# Autodesk Inventor assembly: Framing_For_Roof
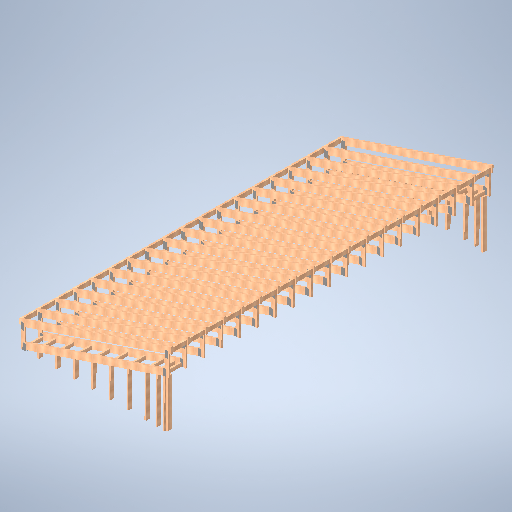
[picture p0: Inventor's stored thumbnail of the model, 512x512]
Saved by Autodesk Inventor 2025.1 (Build 291241020, 241B)
## iProperties
Created: 2024-10-03
Part Number: Framing_For_Roof
Document SubType Name: Assembly
Designer: Tom
Author: Tom
## Documents named in this file (17)
- C:\Users\Tom\Documents\Inventor\Mobility\Additional_Building\Framing_For_Roof.iam
- C:\Users\Tom\Documents\Inventor\Mobility\Additional_Building\Truss.iam
- C:\Users\Tom\Documents\Inventor\Mobility\Additional_Building\Stud_With_Height_5.047_Inches.ipt
- C:\Users\Tom\Documents\Inventor\Mobility\Additional_Building\Stud_With_Height_10.386_Inches.ipt
- C:\Users\Tom\Documents\Inventor\Mobility\Additional_Building\Stud_With_Height_15.724_Inches.ipt
- C:\Users\Tom\Documents\Inventor\Mobility\Additional_Building\Stud_With_Height_21.063_Inches.ipt
- C:\Users\Tom\Documents\Inventor\Mobility\Additional_Building\Stud_With_Height_26.401_Inches.ipt
- C:\Users\Tom\Documents\Inventor\Mobility\Additional_Building\Stud_With_Height_31.740_Inches.ipt
- C:\Users\Tom\Documents\Inventor\Mobility\Additional_Building\Stud_With_Height_37.078_Inches.ipt
- C:\Users\Tom\Documents\Inventor\Mobility\Additional_Building\Stud_With_Height_40.373_Inches.ipt
- C:\Users\Tom\Documents\Inventor\Mobility\Additional_Building\Stud_With_Height_42.5_Inches.ipt
- C:\Users\Tom\Documents\Inventor\Mobility\Additional_Building\Stud_With_Height_42.5_Inches_And_Cut.ipt
- C:\Users\Tom\Documents\Inventor\Mobility\Additional_Building\Subfascia_With_Dimensions_4.023_x_13.75_Inches.ipt
- C:\Users\Tom\Documents\Inventor\Mobility\Additional_Building\Subfascia_With_Dimensions_4.023_x_14.5_Inches.ipt
- C:\Users\Tom\Documents\Inventor\Mobility\Additional_Building\Subfascia_With_Dimensions_3.725_x_13.75_Inches.ipt
- C:\Users\Tom\Documents\Inventor\Mobility\Additional_Building\Subfascia_With_Dimensions_3.725_x_14.5_Inches.ipt
- C:\Users\Tom\Documents\Inventor\Mobility\Additional_Building\Support_For_Ceiling.ipt
## Components (95 placed, 16 different names)
1. Subfascia_With_Dimensions_4.023_x_13.75_Inches:1 — Mate:5, Flush:30, Flush:31
2. Subfascia_With_Dimensions_4.023_x_13.75_Inches:2 — Mate:7, Flush:35, Flush:36
3. Subfascia_With_Dimensions_3.725_x_13.75_Inches:1 — Mate:8, Flush:37, Flush:38
4. Subfascia_With_Dimensions_3.725_x_13.75_Inches:2 — Mate:10, Flush:41, Flush:42
5. Truss:1 [sub-assembly] — Mate:10, Flush:41, Flush:42
6. Truss:2 [sub-assembly] — Flush:1, Flush:2, Flush:3, Flush:4, Flush:5, Flush:6, Flush:8, Flush:9, Flush:11, Flush:12, Flush:14, Flush:15, Flush:17, Flush:18, Flush:20, Flush:21, Flush:23, Flush:24, Flush:26, Mate:2, Flush:28, Mate:3, Mate:5, Flush:30, Flush:31, Flush:32, Mate:11, Flush:44, Mate:12, Mate:13, Flush:46, Mate:14, Flush:48, Mate:15, Flush:50, Mate:16, Flush:52, Mate:17, Flush:54, Mate:18, Flush:56, Mate:19, Flush:58, Mate:20, Flush:60, Mate:21, Flush:62, Flush:65
7. Truss:3 [sub-assembly] — Flush:1, Flush:2, Flush:32, Mate:6, Flush:33, Flush:34, Mate:8, Flush:37, Flush:38
8. Truss:4 [sub-assembly] — Mate:9, Flush:39, Flush:40
9. Truss:5 [sub-assembly]
10. Truss:6 [sub-assembly]
11. Truss:7 [sub-assembly]
12. Truss:8 [sub-assembly]
13. Truss:9 [sub-assembly]
14. Truss:10 [sub-assembly]
15. Truss:11 [sub-assembly]
16. Truss:12 [sub-assembly]
17. Truss:13 [sub-assembly]
18. Truss:14 [sub-assembly]
19. Truss:15 [sub-assembly]
20. Truss:16 [sub-assembly]
21. Truss:17 [sub-assembly]
22. Truss:18 [sub-assembly]
23. Truss:19 [sub-assembly] — Mate:7, Flush:35, Flush:36
24. Subfascia_With_Dimensions_4.023_x_14.5_Inches:1 — Mate:6, Flush:33, Flush:34
25. Subfascia_With_Dimensions_4.023_x_14.5_Inches:2
26. Subfascia_With_Dimensions_4.023_x_14.5_Inches:3
27. Subfascia_With_Dimensions_4.023_x_14.5_Inches:4
28. Subfascia_With_Dimensions_4.023_x_14.5_Inches:5
29. Subfascia_With_Dimensions_4.023_x_14.5_Inches:6
30. Subfascia_With_Dimensions_4.023_x_14.5_Inches:7
31. Subfascia_With_Dimensions_4.023_x_14.5_Inches:8
32. Subfascia_With_Dimensions_4.023_x_14.5_Inches:9
33. Subfascia_With_Dimensions_4.023_x_14.5_Inches:10
34. Subfascia_With_Dimensions_4.023_x_14.5_Inches:11
35. Subfascia_With_Dimensions_4.023_x_14.5_Inches:12
36. Subfascia_With_Dimensions_4.023_x_14.5_Inches:13
37. Subfascia_With_Dimensions_4.023_x_14.5_Inches:14
38. Subfascia_With_Dimensions_4.023_x_14.5_Inches:15
39. Subfascia_With_Dimensions_4.023_x_14.5_Inches:16
40. Subfascia_With_Dimensions_3.725_x_14.5_Inches:1 — Mate:9, Flush:39, Flush:40
41. Subfascia_With_Dimensions_3.725_x_14.5_Inches:2
42. Subfascia_With_Dimensions_3.725_x_14.5_Inches:3
43. Subfascia_With_Dimensions_3.725_x_14.5_Inches:4
44. Subfascia_With_Dimensions_3.725_x_14.5_Inches:5
45. Subfascia_With_Dimensions_3.725_x_14.5_Inches:6
46. Subfascia_With_Dimensions_3.725_x_14.5_Inches:7
47. Subfascia_With_Dimensions_3.725_x_14.5_Inches:8
48. Subfascia_With_Dimensions_3.725_x_14.5_Inches:9
49. Subfascia_With_Dimensions_3.725_x_14.5_Inches:10
50. Subfascia_With_Dimensions_3.725_x_14.5_Inches:11
51. Subfascia_With_Dimensions_3.725_x_14.5_Inches:12
52. Subfascia_With_Dimensions_3.725_x_14.5_Inches:13
53. Subfascia_With_Dimensions_3.725_x_14.5_Inches:14
54. Subfascia_With_Dimensions_3.725_x_14.5_Inches:15
55. Subfascia_With_Dimensions_3.725_x_14.5_Inches:16
56. Support_For_Ceiling:1 — Mate:11, Flush:44, Mate:12
57. Support_For_Ceiling:2 — Mate:13, Flush:45, Flush:46
58. Support_For_Ceiling:3 — Mate:14, Flush:47, Flush:48
59. Support_For_Ceiling:4 — Mate:15, Flush:49, Flush:50
60. Support_For_Ceiling:5 — Mate:16, Flush:51, Flush:52
61. Support_For_Ceiling:6 — Mate:17, Flush:53, Flush:54
62. Support_For_Ceiling:7 — Mate:18, Flush:55, Flush:56
63. Support_For_Ceiling:8 — Mate:19, Flush:57, Flush:58
64. Support_For_Ceiling:9 — Mate:20, Flush:59, Flush:60
65. Support_For_Ceiling:10 — Mate:21, Flush:61, Flush:62
66. Support_For_Ceiling:11
67. Support_For_Ceiling:12
68. Support_For_Ceiling:13
69. Support_For_Ceiling:14
70. Support_For_Ceiling:15
71. Support_For_Ceiling:16
72. Support_For_Ceiling:17
73. Support_For_Ceiling:18
74. Support_For_Ceiling:19
75. Support_For_Ceiling:20
76. Stud_With_Height_5.047_Inches:1 — Flush:3, Flush:4, Flush:5, Flush:7, Flush:45
77. Stud_With_Height_10.386_Inches:1 — Flush:6, Flush:7, Flush:8, Flush:10, Flush:47
78. Stud_With_Height_15.724_Inches:1 — Flush:9, Flush:10, Flush:11, Flush:13, Flush:49
79. Stud_With_Height_21.063_Inches:1 — Flush:12, Flush:13, Flush:14, Flush:16, Flush:51
80. Stud_With_Height_26.401_Inches:1 — Flush:15, Flush:16, Flush:17, Flush:19, Flush:53
81. Stud_With_Height_31.740_Inches:1 — Flush:18, Flush:19, Flush:20, Flush:22, Flush:55
82. Stud_With_Height_37.078_Inches:1 — Flush:21, Flush:22, Flush:23, Flush:25, Flush:57
83. Stud_With_Height_40.373_Inches:1 — Flush:24, Flush:25, Flush:26, Flush:59, Flush:63
84. Stud_With_Height_42.5_Inches_And_Cut:1 — Mate:2, Flush:28, Mate:4, Flush:61, Flush:64, Flush:65
85. Stud_With_Height_5.047_Inches:2
86. Stud_With_Height_10.386_Inches:2
87. Stud_With_Height_15.724_Inches:2
88. Stud_With_Height_21.063_Inches:2
89. Stud_With_Height_26.401_Inches:2
90. Stud_With_Height_31.740_Inches:2
91. Stud_With_Height_37.078_Inches:2
92. Stud_With_Height_40.373_Inches:2
93. Stud_With_Height_42.5_Inches_And_Cut:2
94. Stud_With_Height_42.5_Inches:1 — Mate:3, Mate:4, Flush:63, Flush:64
95. Stud_With_Height_42.5_Inches:2
## Component patterns: (2 elements, first: Truss:1), (17 elements, first: Truss:3), (16 elements, first: Subfascia_With_Dimensions_4.023_x_14.5_Inches:1), (16 elements, first: Subfascia_With_Dimensions_3.725_x_14.5_Inches:1), (2 elements, first: Support_For_Ceiling:1 + Support_For_Ceiling:2 + Support_For_Ceiling:3 + Support_For_Ceiling:4 + Support_For_Ceiling:5 + Support_For_Ceiling:6 + Support_For_Ceiling:7 + Support_For_Ceiling:8 + Support_For_Ceiling:9 + Support_For_Ceiling:10), (2 elements, first: Stud_With_Height_5.047_Inches:1 + Stud_With_Height_10.386_Inches:1 + Stud_With_Height_15.724_Inches:1 + Stud_With_Height_21.063_Inches:1 + Stud_With_Height_26.401_Inches:1 + Stud_With_Height_31.740_Inches:1 + Stud_With_Height_37.078_Inches:1 + Stud_With_Height_40.373_Inches:1 + Stud_With_Height_42.5_Inches_And_Cut:1), (2 elements, first: Stud_With_Height_42.5_Inches:1)
## Relationships (82: Flush 62, Mate 20)
- Flush:1: Truss:2 ↔ Truss:3
- Flush:2: Truss:2 ↔ Truss:3
- Flush:3: Truss:2 ↔ Stud_With_Height_5.047_Inches:1
- Flush:4 (374.65 mm): Truss:2 ↔ Stud_With_Height_5.047_Inches:1
- Flush:5: Truss:2 ↔ Stud_With_Height_5.047_Inches:1
- Flush:6: Truss:2 ↔ Stud_With_Height_10.386_Inches:1
- Flush:7 (406.4 mm): Stud_With_Height_5.047_Inches:1 ↔ Stud_With_Height_10.386_Inches:1
- Flush:8: Truss:2 ↔ Stud_With_Height_10.386_Inches:1
- Flush:9: Truss:2 ↔ Stud_With_Height_15.724_Inches:1
- Flush:10 (406.4 mm): Stud_With_Height_10.386_Inches:1 ↔ Stud_With_Height_15.724_Inches:1
- Flush:11: Truss:2 ↔ Stud_With_Height_15.724_Inches:1
- Flush:12: Truss:2 ↔ Stud_With_Height_21.063_Inches:1
- Flush:13 (406.4 mm): Stud_With_Height_15.724_Inches:1 ↔ Stud_With_Height_21.063_Inches:1
- Flush:14: Truss:2 ↔ Stud_With_Height_21.063_Inches:1
- Flush:15: Truss:2 ↔ Stud_With_Height_26.401_Inches:1
- Flush:16 (406.4 mm): Stud_With_Height_21.063_Inches:1 ↔ Stud_With_Height_26.401_Inches:1
- Flush:17: Truss:2 ↔ Stud_With_Height_26.401_Inches:1
- Flush:18: Truss:2 ↔ Stud_With_Height_31.740_Inches:1
- Flush:19 (406.4 mm): Stud_With_Height_26.401_Inches:1 ↔ Stud_With_Height_31.740_Inches:1
- Flush:20: Truss:2 ↔ Stud_With_Height_31.740_Inches:1
- Flush:21: Truss:2 ↔ Stud_With_Height_37.078_Inches:1
- Flush:22 (406.4 mm): Stud_With_Height_31.740_Inches:1 ↔ Stud_With_Height_37.078_Inches:1
- Flush:23: Truss:2 ↔ Stud_With_Height_37.078_Inches:1
- Flush:24: Truss:2 ↔ Stud_With_Height_40.373_Inches:1
- Flush:25 (250.825 mm): Stud_With_Height_37.078_Inches:1 ↔ Stud_With_Height_40.373_Inches:1
- Flush:26: Truss:2 ↔ Stud_With_Height_40.373_Inches:1
- Mate:2: Truss:2 ↔ Stud_With_Height_42.5_Inches_And_Cut:1
- Flush:28: Truss:2 ↔ Stud_With_Height_42.5_Inches_And_Cut:1
- Mate:3: Truss:2 ↔ Stud_With_Height_42.5_Inches:1
- Mate:4: Stud_With_Height_42.5_Inches_And_Cut:1 ↔ Stud_With_Height_42.5_Inches:1
- Mate:5: Subfascia_With_Dimensions_4.023_x_13.75_Inches:1 ↔ Truss:2
- Flush:30: Subfascia_With_Dimensions_4.023_x_13.75_Inches:1 ↔ Truss:2
- Flush:31: Subfascia_With_Dimensions_4.023_x_13.75_Inches:1 ↔ Truss:2
- Flush:32 (387.35 mm): Truss:2 ↔ Truss:3
- Mate:6: Truss:3 ↔ Subfascia_With_Dimensions_4.023_x_14.5_Inches:1
- Flush:33: Truss:3 ↔ Subfascia_With_Dimensions_4.023_x_14.5_Inches:1
- Flush:34: Truss:3 ↔ Subfascia_With_Dimensions_4.023_x_14.5_Inches:1
- Mate:7: Subfascia_With_Dimensions_4.023_x_13.75_Inches:2 ↔ Truss:19
- Flush:35: Subfascia_With_Dimensions_4.023_x_13.75_Inches:2 ↔ Truss:19
- Flush:36: Subfascia_With_Dimensions_4.023_x_13.75_Inches:2 ↔ Truss:19
- Mate:8: Subfascia_With_Dimensions_3.725_x_13.75_Inches:1 ↔ Truss:3
- Flush:37: Subfascia_With_Dimensions_3.725_x_13.75_Inches:1 ↔ Truss:3
- Flush:38 (25.4 mm): Subfascia_With_Dimensions_3.725_x_13.75_Inches:1 ↔ Truss:3
- Mate:9: Truss:4 ↔ Subfascia_With_Dimensions_3.725_x_14.5_Inches:1
- Flush:39: Truss:4 ↔ Subfascia_With_Dimensions_3.725_x_14.5_Inches:1
- Flush:40 (25.4 mm): Truss:4 ↔ Subfascia_With_Dimensions_3.725_x_14.5_Inches:1
- Mate:10: Subfascia_With_Dimensions_3.725_x_13.75_Inches:2 ↔ Truss:1
- Flush:41: Subfascia_With_Dimensions_3.725_x_13.75_Inches:2 ↔ Truss:1
- Flush:42 (25.4 mm): Subfascia_With_Dimensions_3.725_x_13.75_Inches:2 ↔ Truss:1
- Mate:11: Truss:2 ↔ Support_For_Ceiling:1
- Flush:44: Truss:2 ↔ Support_For_Ceiling:1
- Mate:12: Truss:2 ↔ Support_For_Ceiling:1
- Mate:13: Truss:2 ↔ Support_For_Ceiling:2
- Flush:45: Support_For_Ceiling:2 ↔ Stud_With_Height_5.047_Inches:1
- Flush:46: Truss:2 ↔ Support_For_Ceiling:2
- Mate:14: Truss:2 ↔ Support_For_Ceiling:3
- Flush:47: Support_For_Ceiling:3 ↔ Stud_With_Height_10.386_Inches:1
- Flush:48: Truss:2 ↔ Support_For_Ceiling:3
- Mate:15: Truss:2 ↔ Support_For_Ceiling:4
- Flush:49: Support_For_Ceiling:4 ↔ Stud_With_Height_15.724_Inches:1
- Flush:50: Truss:2 ↔ Support_For_Ceiling:4
- Mate:16: Truss:2 ↔ Support_For_Ceiling:5
- Flush:51: Support_For_Ceiling:5 ↔ Stud_With_Height_21.063_Inches:1
- Flush:52: Truss:2 ↔ Support_For_Ceiling:5
- Mate:17: Truss:2 ↔ Support_For_Ceiling:6
- Flush:53: Support_For_Ceiling:6 ↔ Stud_With_Height_26.401_Inches:1
- Flush:54: Truss:2 ↔ Support_For_Ceiling:6
- Mate:18: Truss:2 ↔ Support_For_Ceiling:7
- Flush:55: Support_For_Ceiling:7 ↔ Stud_With_Height_31.740_Inches:1
- Flush:56: Truss:2 ↔ Support_For_Ceiling:7
- Mate:19: Truss:2 ↔ Support_For_Ceiling:8
- Flush:57: Support_For_Ceiling:8 ↔ Stud_With_Height_37.078_Inches:1
- Flush:58: Truss:2 ↔ Support_For_Ceiling:8
- Mate:20: Truss:2 ↔ Support_For_Ceiling:9
- Flush:59: Support_For_Ceiling:9 ↔ Stud_With_Height_40.373_Inches:1
- Flush:60: Truss:2 ↔ Support_For_Ceiling:9
- Mate:21: Truss:2 ↔ Support_For_Ceiling:10
- Flush:61: Support_For_Ceiling:10 ↔ Stud_With_Height_42.5_Inches_And_Cut:1
- Flush:62: Truss:2 ↔ Support_For_Ceiling:10
- Flush:63: Stud_With_Height_40.373_Inches:1 ↔ Stud_With_Height_42.5_Inches:1
- Flush:64: Stud_With_Height_42.5_Inches_And_Cut:1 ↔ Stud_With_Height_42.5_Inches:1
- Flush:65: Truss:2 ↔ Stud_With_Height_42.5_Inches_And_Cut:1
